# Autodesk Inventor assembly: fc16-044
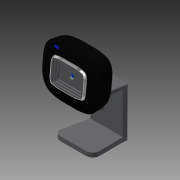
[picture p0: Inventor's stored thumbnail of the model, 180x180]
Saved by Autodesk Inventor 2016 SP1 (Build 200210100, 210)
## iProperties
Category: Electronics
Company: Autodesk Inc.
Created: 2015-11-24
Part Number: fc16-044
Document SubType Name: Assembly
Designer: Autodesk Inc.
Catalog Web Link: http://www.microsoft.com/hardware/en-ca/p/lifecam-hd-3000
Vendor: Microsoft Inc.
Author: Autodesk Inc.
Keywords: FIRSTChoice
## Documents named in this file (3)
- D:\FIRST\FRC KOP 2016\FRC FIRSTChoice 2016\Electronics\fc16-044_Camera.iam
- D:\FIRST\FRC KOP 2016\FRC FIRSTChoice 2016\Controls\Parts\CS_Camera_HD3000.ipt
- D:\FIRST\FRC KOP 2016\FRC FIRSTChoice 2016\Controls\Parts\CS_Camera_HD3000_Base_01.ipt
## Components (2 placed, 2 different names)
1. CS_Camera_HD3000:1 — Mate:1, Mate:2
2. CS_Camera_HD3000_Base_01:1 — Mate:1, Mate:2
## Relationships (2: Mate 2)
- Mate:1: CS_Camera_HD3000:1 ↔ CS_Camera_HD3000_Base_01:1
- Mate:2: CS_Camera_HD3000:1 ↔ CS_Camera_HD3000_Base_01:1
